# Autodesk Inventor assembly: Hepheaestes38_Case_Assy
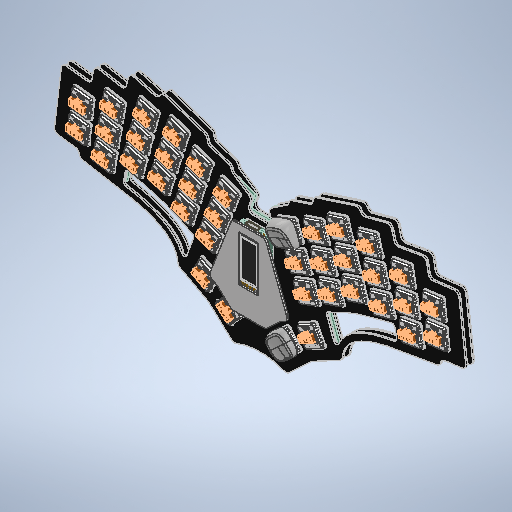
[picture p0: Inventor's stored thumbnail of the model, 512x512]
Saved by Autodesk Inventor 2025 (Build 290162000, 162)
## iProperties
Company: Kicad
Created: 2025-04-19
Part Number: Hepheaestes38_Case_Assy
Description: KiCad electronic assembly
Document SubType Name: Assembly
Designer: User
Authority: Unknown
Sending System: KiCad to STEP converter
Preprocessor: Open CASCADE STEP processor 7.8
Title: Hepheaestes38_PCB.step
Author: Pcbnew
## Documents named in this file (11)
- C:\Users\User\Hephaestes38-zmk\PCB, Case\New folder\Hepheaestes38_Case_Assy.iam
- C:\Users\User\Hephaestes38-zmk\PCB, Case\kicad PCB files\Hepheaestes38_PCB\Hepheaestes38_PCB_PCB.ipt
- C:\Users\User\Documents\3d Printing\Hot Swap Socket negative.ipt
- C:\Users\User\Downloads\kailh-choc-low-profile-switch-1.snapshot.3\Kailh Choc Low Profile Switch\Kailh Choc Low Profile Switch.ipt
- C:\Users\User\Hephaestes38-zmk\PCB, Case\New folder\Acrylic Top.ipt
- C:\Users\User\Hephaestes38-zmk\PCB, Case\New folder\Acrylic bottom.ipt
- C:\Users\User\Downloads\nice!nano v2\nice!nano v2.iam
- C:\Users\User\Downloads\nice!view.ipt
- C:\Users\User\Hephaestes38-zmk\PCB, Case\New folder\Screen Cover.ipt
- C:\Users\User\Downloads\KLP_Lame_Thumb\KLP_Lame_Thumb.ipt
- C:\Users\User\Downloads\KLP_Lame_Saddle_Tilted\KLP_Lame_Saddle_Tilted.ipt
## Components (84 placed, 10 different names)
1. 1 — Mate:35, Mate:2, Mate:34, Angle:18, Mate:36, Angle:19, Mate:37, Mate:38, Mate:39, Mate:40, Mate:41, Mate:42, Mate:43, Mate:44, Mate:45, Mate:46, Mate:47, Mate:48, Mate:49, Mate:50, Mate:51, Mate:52, Mate:53, Mate:54, Mate:55, Mate:56, Mate:57, Mate:58, Mate:59, Mate:60, Mate:61, Mate:62, Mate:63, Mate:64, Mate:65, Mate:66, Angle:20, Angle:21, Angle:22, Angle:23, Angle:24, Angle:25, Angle:26, Angle:27, Angle:28, Angle:29, Angle:30, Angle:31, Angle:32, Angle:33, Angle:34, Mate:67, Mate:68, Mate:69, Mate:70, Mate:71, Mate:72, Mate:73, Mate:74, Mate:75, Mate:76, Mate:77, Mate:78, Mate:79, Mate:80, Mate:81, Mate:82, Mate:83, Mate:84, Mate:85, Mate:86, Mate:87, Mate:88, Mate:89, Mate:90, Mate:91, Mate:92, Mate:93, Mate:94, Mate:95, Mate:96, Angle:35, Angle:36, Angle:37, Angle:38, Angle:39, Angle:40, Angle:41, Angle:42, Angle:43, Angle:44, Angle:45, Angle:46, Angle:47, Angle:48, Angle:49, Flush:3, Mate:101, Mate:102, Flush:4, Mate:103, Mate:104
2. Hot Swap Socket negative:7 — Mate:42, Mate:56, Angle:31
3. Hot Swap Socket negative:8 — Mate:43, Mate:57, Angle:32
4. Hot Swap Socket negative:9 — Mate:44, Mate:58, Angle:33
5. Hot Swap Socket negative:11 — Mate:45, Mate:59, Angle:34
6. Kailh Choc Low Profile Switch:9 — Mate:77, Mate:96, Angle:44, Mate:100
7. Kailh Choc Low Profile Switch:10 — Mate:78, Mate:95, Angle:43
8. Kailh Choc Low Profile Switch:11 — Mate:79, Mate:94, Angle:42, Mate:117, Mate:118, Tangent:1
9. Kailh Choc Low Profile Switch:12 — Mate:80, Mate:93, Angle:41
10. Acrylic Top:1 — Mate:97, Mate:98, Mate:99, Flush:1, Flush:2
11. Acrylic bottom:1 — Mate:100, Flush:1, Flush:2
12. nice!nano v2:1 [sub-assembly] — Flush:3, Mate:101, Mate:102
13. nice!view:1 — Flush:4, Mate:103, Mate:104, Mate:105, Mate:106, Mate:107
14. Screen Cover:1 — Mate:105, Mate:106, Mate:107
15. KLP_Lame_Saddle_Tilted:1 — Mate:113, Mate:114
16. KLP_Lame_Thumb:1 — Mate:117, Mate:118, Tangent:1
17. Hot Swap Socket negative:10 — Mate:60, Mate:61, Angle:25
18. Kailh Choc Low Profile Switch:13 — Mate:81, Mate:92, Angle:35, Mate:113, Mate:114
19. Hot Swap Socket negative:17
20. Kailh Choc Low Profile Switch:19
21. Hot Swap Socket negative:18
22. Kailh Choc Low Profile Switch:20
23. Hot Swap Socket negative:12 — Mate:46, Mate:62, Angle:24
24. Kailh Choc Low Profile Switch:14 — Mate:82, Mate:91, Angle:36, Mate:97
25. Hot Swap Socket negative:19
26. Kailh Choc Low Profile Switch:21
27. Hot Swap Socket negative:20
28. Kailh Choc Low Profile Switch:22
29. Hot Swap Socket negative:13 — Mate:47, Mate:63, Angle:23
30. Kailh Choc Low Profile Switch:15 — Mate:83, Mate:90, Angle:37
31. Hot Swap Socket negative:21
32. Kailh Choc Low Profile Switch:23
33. Hot Swap Socket negative:22
34. Kailh Choc Low Profile Switch:24
35. Hot Swap Socket negative:14 — Mate:48, Mate:64, Angle:22
36. Kailh Choc Low Profile Switch:16 — Mate:84, Mate:89, Angle:38
37. Hot Swap Socket negative:23
38. Kailh Choc Low Profile Switch:25
39. Hot Swap Socket negative:24
40. Kailh Choc Low Profile Switch:26
41. Hot Swap Socket negative:15 — Mate:49, Mate:65, Angle:21
42. Kailh Choc Low Profile Switch:17 — Mate:85, Mate:88, Angle:39
43. Hot Swap Socket negative:25
44. Kailh Choc Low Profile Switch:27
45. Hot Swap Socket negative:26
46. Kailh Choc Low Profile Switch:28
47. Hot Swap Socket negative:16 — Mate:50, Mate:66, Angle:20
48. Kailh Choc Low Profile Switch:18 — Mate:86, Mate:87, Angle:40
49. Hot Swap Socket negative:27
50. Kailh Choc Low Profile Switch:29
51. Hot Swap Socket negative:1 — Mate:35, Mate:2, Angle:18
52. Kailh Choc Low Profile Switch:1 — Mate:34, Mate:36, Angle:19, Mate:98, Mate:99
53. Hot Swap Socket negative:28
54. Kailh Choc Low Profile Switch:2
55. Hot Swap Socket negative:29
56. Kailh Choc Low Profile Switch:3
57. Hot Swap Socket negative:2 — Mate:37, Mate:51, Angle:26
58. Kailh Choc Low Profile Switch:5 — Mate:68, Mate:72, Angle:45
59. Hot Swap Socket negative:30
60. Kailh Choc Low Profile Switch:30
61. Hot Swap Socket negative:31
62. Kailh Choc Low Profile Switch:31
63. Hot Swap Socket negative:3 — Mate:38, Mate:52, Angle:27
64. Kailh Choc Low Profile Switch:4 — Mate:67, Mate:73, Angle:46
65. Hot Swap Socket negative:32
66. Kailh Choc Low Profile Switch:32
67. Hot Swap Socket negative:33
68. Kailh Choc Low Profile Switch:33
69. Hot Swap Socket negative:4 — Mate:39, Mate:53, Angle:28
70. Kailh Choc Low Profile Switch:6 — Mate:69, Mate:74, Angle:47
71. Hot Swap Socket negative:34
72. Kailh Choc Low Profile Switch:34
73. Hot Swap Socket negative:35
74. Kailh Choc Low Profile Switch:35
75. Hot Swap Socket negative:5 — Mate:40, Mate:54, Angle:29
76. Kailh Choc Low Profile Switch:7 — Mate:70, Mate:75, Angle:48
77. Hot Swap Socket negative:36
78. Kailh Choc Low Profile Switch:36
79. Hot Swap Socket negative:37
80. Kailh Choc Low Profile Switch:37
81. Hot Swap Socket negative:6 — Mate:41, Mate:55, Angle:30
82. Kailh Choc Low Profile Switch:8 — Mate:71, Mate:76, Angle:49
83. Hot Swap Socket negative:38
84. Kailh Choc Low Profile Switch:38
## Component patterns: (3 elements, first: Hot Swap Socket negative:10 + Kailh Choc Low Profile Switch:13), (3 elements, first: Hot Swap Socket negative:12 + Kailh Choc Low Profile Switch:14), (3 elements, first: Hot Swap Socket negative:13 + Kailh Choc Low Profile Switch:15), (3 elements, first: Hot Swap Socket negative:14 + Kailh Choc Low Profile Switch:16), (3 elements, first: Hot Swap Socket negative:15 + Kailh Choc Low Profile Switch:17), (2 elements, first: Hot Swap Socket negative:16 + Kailh Choc Low Profile Switch:18), (3 elements, first: Hot Swap Socket negative:1 + Kailh Choc Low Profile Switch:1), (3 elements, first: Hot Swap Socket negative:2 + Kailh Choc Low Profile Switch:5), (3 elements, first: Hot Swap Socket negative:3 + Kailh Choc Low Profile Switch:4), (3 elements, first: Hot Swap Socket negative:4 + Kailh Choc Low Profile Switch:6), (3 elements, first: Hot Swap Socket negative:5 + Kailh Choc Low Profile Switch:7), (2 elements, first: Hot Swap Socket negative:6 + Kailh Choc Low Profile Switch:8)
## Relationships (116: Mate 79, Angle 32, Flush 4, Tangent 1)
- Mate:35: 1 ↔ Hot Swap Socket negative:1
- Mate:2: 1 ↔ Hot Swap Socket negative:1
- Mate:34: 1 ↔ Kailh Choc Low Profile Switch:1
- Angle:18 (0 deg): 1 ↔ Hot Swap Socket negative:1
- Mate:36: 1 ↔ Kailh Choc Low Profile Switch:1
- Angle:19 (0 deg): 1 ↔ Kailh Choc Low Profile Switch:1
- Mate:37: 1 ↔ Hot Swap Socket negative:2
- Mate:38: 1 ↔ Hot Swap Socket negative:3
- Mate:39: 1 ↔ Hot Swap Socket negative:4
- Mate:40: 1 ↔ Hot Swap Socket negative:5
- Mate:41: 1 ↔ Hot Swap Socket negative:6
- Mate:42: 1 ↔ Hot Swap Socket negative:7
- Mate:43: 1 ↔ Hot Swap Socket negative:8
- Mate:44: 1 ↔ Hot Swap Socket negative:9
- Mate:45: 1 ↔ Hot Swap Socket negative:11
- Mate:46: 1 ↔ Hot Swap Socket negative:12
- Mate:47: 1 ↔ Hot Swap Socket negative:13
- Mate:48: 1 ↔ Hot Swap Socket negative:14
- Mate:49: 1 ↔ Hot Swap Socket negative:15
- Mate:50: 1 ↔ Hot Swap Socket negative:16
- Mate:51: 1 ↔ Hot Swap Socket negative:2
- Mate:52: 1 ↔ Hot Swap Socket negative:3
- Mate:53: 1 ↔ Hot Swap Socket negative:4
- Mate:54: 1 ↔ Hot Swap Socket negative:5
- Mate:55: 1 ↔ Hot Swap Socket negative:6
- Mate:56: 1 ↔ Hot Swap Socket negative:7
- Mate:57: 1 ↔ Hot Swap Socket negative:8
- Mate:58: 1 ↔ Hot Swap Socket negative:9
- Mate:59: 1 ↔ Hot Swap Socket negative:11
- Mate:60: 1 ↔ Hot Swap Socket negative:10
- Mate:61: 1 ↔ Hot Swap Socket negative:10
- Mate:62: 1 ↔ Hot Swap Socket negative:12
- Mate:63: 1 ↔ Hot Swap Socket negative:13
- Mate:64: 1 ↔ Hot Swap Socket negative:14
- Mate:65: 1 ↔ Hot Swap Socket negative:15
- Mate:66: 1 ↔ Hot Swap Socket negative:16
- Angle:20 (0 deg): 1 ↔ Hot Swap Socket negative:16
- Angle:21 (0 deg): 1 ↔ Hot Swap Socket negative:15
- Angle:22 (0 deg): 1 ↔ Hot Swap Socket negative:14
- Angle:23 (0 deg): 1 ↔ Hot Swap Socket negative:13
- Angle:24 (0 deg): 1 ↔ Hot Swap Socket negative:12
- Angle:25 (0 deg): 1 ↔ Hot Swap Socket negative:10
- Angle:26 (0 deg): 1 ↔ Hot Swap Socket negative:2
- Angle:27 (0 deg): 1 ↔ Hot Swap Socket negative:3
- Angle:28 (0 deg): 1 ↔ Hot Swap Socket negative:4
- Angle:29 (0 deg): 1 ↔ Hot Swap Socket negative:5
- Angle:30 (0 deg): 1 ↔ Hot Swap Socket negative:6
- Angle:31 (0 deg): 1 ↔ Hot Swap Socket negative:7
- Angle:32 (0 deg): 1 ↔ Hot Swap Socket negative:8
- Angle:33 (0 deg): 1 ↔ Hot Swap Socket negative:9
- Angle:34 (0 deg): 1 ↔ Hot Swap Socket negative:11
- Mate:67: 1 ↔ Kailh Choc Low Profile Switch:4
- Mate:68: 1 ↔ Kailh Choc Low Profile Switch:5
- Mate:69: 1 ↔ Kailh Choc Low Profile Switch:6
- Mate:70: 1 ↔ Kailh Choc Low Profile Switch:7
- Mate:71: 1 ↔ Kailh Choc Low Profile Switch:8
- Mate:72: 1 ↔ Kailh Choc Low Profile Switch:5
- Mate:73: 1 ↔ Kailh Choc Low Profile Switch:4
- Mate:74: 1 ↔ Kailh Choc Low Profile Switch:6
- Mate:75: 1 ↔ Kailh Choc Low Profile Switch:7
- Mate:76: 1 ↔ Kailh Choc Low Profile Switch:8
- Mate:77: 1 ↔ Kailh Choc Low Profile Switch:9
- Mate:78: 1 ↔ Kailh Choc Low Profile Switch:10
- Mate:79: 1 ↔ Kailh Choc Low Profile Switch:11
- Mate:80: 1 ↔ Kailh Choc Low Profile Switch:12
- Mate:81: 1 ↔ Kailh Choc Low Profile Switch:13
- Mate:82: 1 ↔ Kailh Choc Low Profile Switch:14
- Mate:83: 1 ↔ Kailh Choc Low Profile Switch:15
- Mate:84: 1 ↔ Kailh Choc Low Profile Switch:16
- Mate:85: 1 ↔ Kailh Choc Low Profile Switch:17
- Mate:86: 1 ↔ Kailh Choc Low Profile Switch:18
- Mate:87: 1 ↔ Kailh Choc Low Profile Switch:18
- Mate:88: 1 ↔ Kailh Choc Low Profile Switch:17
- Mate:89: 1 ↔ Kailh Choc Low Profile Switch:16
- Mate:90: 1 ↔ Kailh Choc Low Profile Switch:15
- Mate:91: 1 ↔ Kailh Choc Low Profile Switch:14
- Mate:92: 1 ↔ Kailh Choc Low Profile Switch:13
- Mate:93: 1 ↔ Kailh Choc Low Profile Switch:12
- Mate:94: 1 ↔ Kailh Choc Low Profile Switch:11
- Mate:95: 1 ↔ Kailh Choc Low Profile Switch:10
- Mate:96: 1 ↔ Kailh Choc Low Profile Switch:9
- Angle:35 (0 deg): 1 ↔ Kailh Choc Low Profile Switch:13
- Angle:36 (0 deg): 1 ↔ Kailh Choc Low Profile Switch:14
- Angle:37 (0 deg): 1 ↔ Kailh Choc Low Profile Switch:15
- Angle:38 (0 deg): 1 ↔ Kailh Choc Low Profile Switch:16
- Angle:39 (0 deg): 1 ↔ Kailh Choc Low Profile Switch:17
- Angle:40 (0 deg): 1 ↔ Kailh Choc Low Profile Switch:18
- Angle:41 (0 deg): 1 ↔ Kailh Choc Low Profile Switch:12
- Angle:42 (0 deg): 1 ↔ Kailh Choc Low Profile Switch:11
- Angle:43 (0 deg): 1 ↔ Kailh Choc Low Profile Switch:10
- Angle:44 (0 deg): 1 ↔ Kailh Choc Low Profile Switch:9
- Angle:45 (0 deg): 1 ↔ Kailh Choc Low Profile Switch:5
- Angle:46 (0 deg): 1 ↔ Kailh Choc Low Profile Switch:4
- Angle:47 (0 deg): 1 ↔ Kailh Choc Low Profile Switch:6
- Angle:48 (0 deg): 1 ↔ Kailh Choc Low Profile Switch:7
- Angle:49 (0 deg): 1 ↔ Kailh Choc Low Profile Switch:8
- Mate:97: Acrylic Top:1 ↔ Kailh Choc Low Profile Switch:14
- Mate:98: Acrylic Top:1 ↔ Kailh Choc Low Profile Switch:1
- Mate:99: Acrylic Top:1 ↔ Kailh Choc Low Profile Switch:1
- Mate:100: Kailh Choc Low Profile Switch:9 ↔ Acrylic bottom:1
- Flush:1: Acrylic Top:1 ↔ Acrylic bottom:1
- Flush:2: Acrylic Top:1 ↔ Acrylic bottom:1
- Flush:3 (-7 mm): 1 ↔ nice!nano v2:1
- Mate:101: 1 ↔ nice!nano v2:1
- Mate:102: 1 ↔ nice!nano v2:1
- Flush:4 (-10 mm): 1 ↔ nice!view:1
- Mate:103: 1 ↔ nice!view:1
- Mate:104: 1 ↔ nice!view:1
- Mate:105: nice!view:1 ↔ Screen Cover:1
- Mate:106: nice!view:1 ↔ Screen Cover:1
- Mate:107: nice!view:1 ↔ Screen Cover:1
- Mate:113: KLP_Lame_Saddle_Tilted:1 ↔ Kailh Choc Low Profile Switch:13
- Mate:114: KLP_Lame_Saddle_Tilted:1 ↔ Kailh Choc Low Profile Switch:13
- Mate:117: Kailh Choc Low Profile Switch:11 ↔ KLP_Lame_Thumb:1
- Mate:118: Kailh Choc Low Profile Switch:11 ↔ KLP_Lame_Thumb:1
- Tangent:1: Kailh Choc Low Profile Switch:11 ↔ KLP_Lame_Thumb:1
